# Autodesk Inventor assembly: Assenbly1
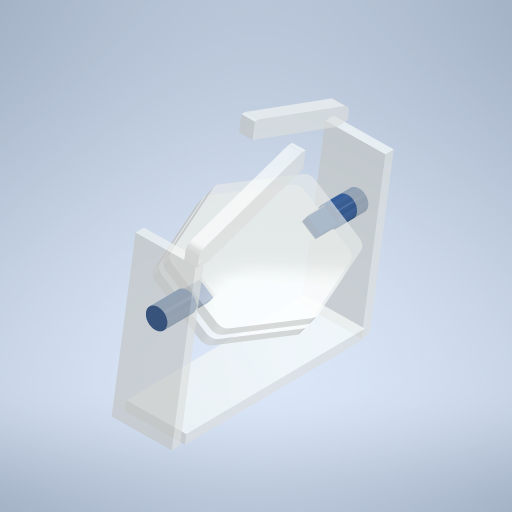
[picture p0: Inventor's stored thumbnail of the model, 512x512]
Saved by Autodesk Inventor 2023.1 (Build 271208000, 208)
## iProperties
Created: 2022-10-25
Part Number: Assenbly1
Document SubType Name: Assembly
Designer: jshin23
Author: jshin23
## Documents named in this file (6)
- C:\Users\jshin23\Desktop\Kids Toy\Assenbly1.iam
- C:\Users\jshin23\Desktop\Kids Toy\Part1 x 2.ipt
- C:\Users\jshin23\Desktop\Kids Toy\Part2 x 1.ipt
- C:\Users\jshin23\Desktop\Kids Toy\Part4 x 2.ipt
- C:\Users\jshin23\Desktop\Kids Toy\Part6 x 2.ipt
- C:\Users\jshin23\Desktop\Kids Toy\Part3 x 2.ipt
## Components (9 placed, 5 different names)
1. Part1 x 2:1 — Mate:1, Flush:1, Flush:2, Mate:2, Mate:6, Mate:7
2. Part1 x 2:2 — Mate:1, Flush:1, Flush:2, Mate:3, Mate:4, Mate:5
3. Part4 x 2:1 — Mate:20, Flush:7, Flush:8, Flush:11, Mate:23
4. Part4 x 2:2 — Mate:21, Flush:10, Flush:11, Flush:12, Mate:23
5. Part6 x 2:1 — Mate:4, Mate:5, Mate:6, Insert:1
6. Part6 x 2:2 — Mate:2, Mate:3, Mate:7, Mate:26
7. Part3 x 2:1 — Mate:21, Flush:10, Flush:12, Insert:1
8. Part3 x 2:2 — Mate:20, Flush:7, Flush:8, Mate:25, Flush:13, Mate:26, Flush:14
9. Part2 x 1:1 — Mate:25, Flush:13, Flush:14
## Relationships (22: Mate 12, Flush 9, Insert 1)
- Mate:1: Part1 x 2:1 ↔ Part1 x 2:2
- Flush:1: Part1 x 2:1 ↔ Part1 x 2:2
- Flush:2: Part1 x 2:1 ↔ Part1 x 2:2
- Mate:2: Part1 x 2:1 ↔ Part6 x 2:2
- Mate:3: Part1 x 2:2 ↔ Part6 x 2:2
- Mate:4: Part1 x 2:2 ↔ Part6 x 2:1
- Mate:5: Part1 x 2:2 ↔ Part6 x 2:1
- Mate:6: Part1 x 2:1 ↔ Part6 x 2:1
- Mate:7: Part1 x 2:1 ↔ Part6 x 2:2
- Mate:20: Part4 x 2:1 ↔ Part3 x 2:2
- Flush:7: Part4 x 2:1 ↔ Part3 x 2:2
- Flush:8: Part4 x 2:1 ↔ Part3 x 2:2
- Mate:21: Part4 x 2:2 ↔ Part3 x 2:1
- Flush:10: Part4 x 2:2 ↔ Part3 x 2:1
- Flush:11: Part4 x 2:1 ↔ Part4 x 2:2
- Flush:12: Part4 x 2:2 ↔ Part3 x 2:1
- Mate:23: Part4 x 2:1 ↔ Part4 x 2:2
- Insert:1 (-20.32 mm): Part6 x 2:1 ↔ Part3 x 2:1
- Mate:25: Part3 x 2:2 ↔ Part2 x 1:1
- Flush:13: Part3 x 2:2 ↔ Part2 x 1:1
- Mate:26: Part6 x 2:2 ↔ Part3 x 2:2
- Flush:14: Part3 x 2:2 ↔ Part2 x 1:1
